# Autodesk Inventor assembly: sunon_fan_red
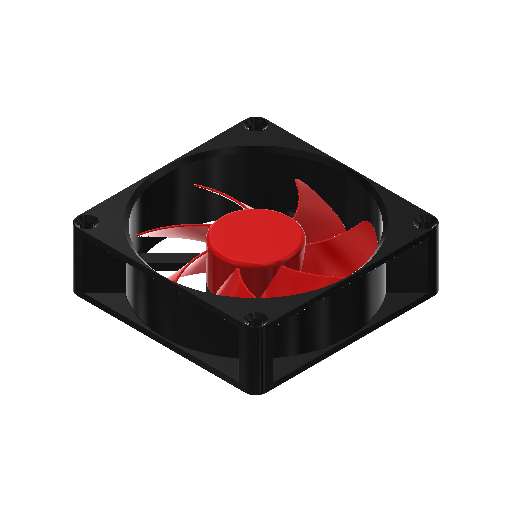
[picture p0: Inventor's stored thumbnail of the model, 512x512]
Saved by Autodesk Inventor 2026.1 (Build 301233000, 233)
## iProperties
Created: 2015-03-08
Part Number: sunon_fan_red
Document SubType Name: Assembly
Designer: Venci
Author: Venci
## Documents named in this file (3)
- C:\Users\Andrzej\OneDrive\_DRIVE_SYNCH_FILES\__ BYTECHLAB PROJECTS\MECH - T-REX 300 – A completely new printer based on a old one\MCAD\1_REV1\__COTS_PARTS\COTS_GENERIC_80mm_fan\COTS_GENERIC_80mm_fan.iam
- C:\Users\Andrzej\OneDrive\_DRIVE_SYNCH_FILES\__ BYTECHLAB PROJECTS\MECH - T-REX 300 – A completely new printer based on a old one\MCAD\1_REV1\__COTS_PARTS\COTS_GENERIC_80mm_fan\sunon_frame.ipt
- C:\Users\Andrzej\OneDrive\_DRIVE_SYNCH_FILES\__ BYTECHLAB PROJECTS\MECH - T-REX 300 – A completely new printer based on a old one\MCAD\1_REV1\__COTS_PARTS\COTS_GENERIC_80mm_fan\sunon_blade_80.ipt
## Components (2 placed, 2 different names)
1. sunon_frame:1 — Insert:1
2. sunon_blade_80:1 — Insert:1
## Relationships (1: Insert 1)
- Insert:1: sunon_frame:1 ↔ sunon_blade_80:1
